# Autodesk Inventor assembly: Assembly1
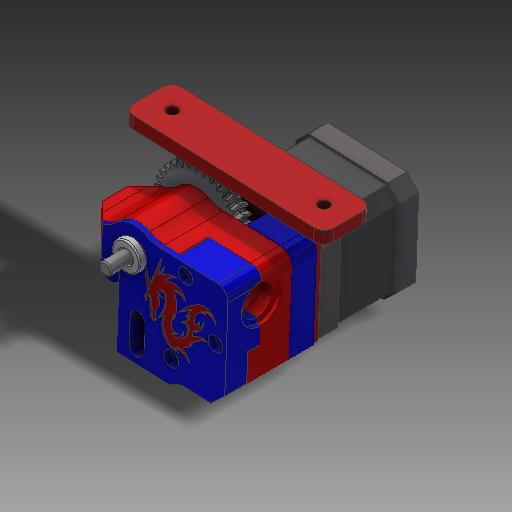
[picture p0: Inventor's stored thumbnail of the model, 512x512]
Saved by Autodesk Inventor 2017.3 (Build 213256000, 256)
## iProperties
Created: 2018-09-06
Part Number: Assembly1
Document SubType Name: Assembly
Designer: Ax
Author: Ax
## iProperties of the stored document PM Wantai 609  Nema 17.ipt
Created: 2015-03-22
Part Number: PM Wantai 609  Nema 17
Material: Generic
Document SubType Name: Modeling
Designer: Ax
Density: 1 g/cm^3
Appearance: Default
Sending System: Autodesk Inventor 2015
Preprocessor: ST-DEVELOPER v15.6
Title: D:\Dropbox\3D parts lib\Inventor\Nema 17s\Wantai 609\PM Wantai 609  Nema 17.stp
Author: Phil
## Documents named in this file (16)
- **C:\Users\Ax\Documents\Inventor\Drakon\Assembly1.iam*LocalDocs*x1hxt1kqvYop2ua0uThhu3lz2Aa*PM Wantai 609  Nema 17.ipt
- C:\Users\Ax\Documents\Inventor\Drakon\Assembly1.iam
- C:\Users\Ax\Documents\Inventor\Drakon\RAMPSDrakon_1.75_Body.ipt
- C:\Users\Ax\Documents\Inventor\Drakon\RAMPSDrakon_1.75_Cover.ipt
- C:\Users\Ax\Documents\Inventor\Drakon\RAMPSDrakon_1.75_Idler.ipt
- C:\Users\Ax\Documents\Inventor\Drakon\RAMPSDrakon_Base.ipt
- C:\Users\Ax\Documents\Inventor\Drakon\RAMPSFrame_Mount.ipt
- C:\Users\Ax\Documents\Inventor\Drakon\RAMPSDrakon_Small_Gear.ipt
- C:\Users\Ax\Documents\Inventor\Drakon\RAMPSDrakon_Large_Gear.ipt
- C:\Users\Ax\Documents\Inventor\Drakon\Library\625ZZ.ipt
- C:\Users\Ax\Documents\Inventor\Drakon\Library\M5x40_Hex_Bolt.ipt
- C:\Users\Ax\Documents\Inventor\Drakon\Library\MK8.ipt
- C:\Users\Ax\Documents\Inventor\Drakon\Library\Drakon_Spindle_Bushing.ipt
- C:\Users\Ax\Documents\Inventor\Drakon\Library\Drakon_1.75_Filament_Guide.ipt
- C:\Users\Ax\Documents\Inventor\Drakon\Assembly1\Design Accelerator\Compress Spring1.iam
- C:\Users\Ax\Documents\Git\Drakon-Extruder\FreeCAD\STEP\PM Wantai 609  Nema 17.stp
## Components (16 placed, 14 different names)
1. Drakon_1.75_Body:1 — Rigid:1, Mate:1, Mate:5, Mate:6, Rotational:4, Mate:10, Mate:11, Mate:12, Mate:13, Mate:14, Rotational:6, Mate:15, Mate:16, Mate:17, Mate:18, Mate:19, Mate:20
2. RAMPSDrakon_1.75_Cover:1 — Rigid:1, Mate:10, Mate:11, Mate:12, Cylindrical:1
3. RAMPSDrakon_1.75_Idler:1 — Rotational:4
4. RAMPSDrakon_Base:1 — Mate:1, Mate:2, Mate:4, Mate:5, Mate:6
5. PM Wantai 609  Nema 17:1 — Rotational:2, Mate:3, Mate:7, Mate:8, Mate:9, Rotational:3
6. RAMPSFrame_Mount:1 — Mate:2, Rotational:2, Mate:3, Mate:4, Mate:7, Mate:8, Mate:9
7. RAMPSDrakon_Small_Gear:1 — Rotational:3, Rotational:6
8. RAMPSDrakon_Large_Gear:1 — Rotational:7, Insert:1
9. 625ZZ:1 — Mate:14, Rotational:7, Mate:15, Rotational:8
10. 625ZZ:2 — Mate:13, Mate:16
11. M5x40_Hex_Bolt:1 — Insert:1, Rigid:2
12. MK8:1 — Rotational:8, Rotational:9
13. Drakon_Spindle_Bushing:1 — Rotational:9
14. Drakon_Spindle_Bushing:2 — Cylindrical:1, Rigid:2
15. Drakon_1.75_Filament_Guide:1 — Mate:17, Mate:18, Mate:19
16. Compress Spring:1 [sub-assembly] — Mate:20
## Relationships (31: Mate 20, RevoluteJoint 7, WeldJoint 2, Insert 1, CylindricalJoint 1)
- Rigid:1 [WeldJoint]: Drakon_1.75_Body:1 ↔ RAMPSDrakon_1.75_Cover:1
- Mate:1: Drakon_1.75_Body:1 ↔ RAMPSDrakon_Base:1
- Mate:2: RAMPSDrakon_Base:1 ↔ RAMPSFrame_Mount:1
- Rotational:2 [RevoluteJoint]: PM Wantai 609  Nema 17:1 ↔ RAMPSFrame_Mount:1
- Mate:3: PM Wantai 609  Nema 17:1 ↔ RAMPSFrame_Mount:1
- Mate:4: RAMPSDrakon_Base:1 ↔ RAMPSFrame_Mount:1
- Mate:5: Drakon_1.75_Body:1 ↔ RAMPSDrakon_Base:1
- Mate:6: Drakon_1.75_Body:1 ↔ RAMPSDrakon_Base:1
- Mate:7: PM Wantai 609  Nema 17:1 ↔ RAMPSFrame_Mount:1
- Mate:8: PM Wantai 609  Nema 17:1 ↔ RAMPSFrame_Mount:1
- Mate:9: PM Wantai 609  Nema 17:1 ↔ RAMPSFrame_Mount:1
- Rotational:3 [RevoluteJoint] (-6.35 mm): PM Wantai 609  Nema 17:1 ↔ RAMPSDrakon_Small_Gear:1
- Rotational:4 [RevoluteJoint]: Drakon_1.75_Body:1 ↔ RAMPSDrakon_1.75_Idler:1
- Mate:10: Drakon_1.75_Body:1 ↔ RAMPSDrakon_1.75_Cover:1
- Mate:11: Drakon_1.75_Body:1 ↔ RAMPSDrakon_1.75_Cover:1
- Mate:12: Drakon_1.75_Body:1 ↔ RAMPSDrakon_1.75_Cover:1
- Mate:13: Drakon_1.75_Body:1 ↔ 625ZZ:2
- Mate:14: Drakon_1.75_Body:1 ↔ 625ZZ:1
- Rotational:6 [RevoluteJoint] (-1.25 mm): Drakon_1.75_Body:1 ↔ RAMPSDrakon_Small_Gear:1
- Rotational:7 [RevoluteJoint] (-1.5 mm): RAMPSDrakon_Large_Gear:1 ↔ 625ZZ:1
- Insert:1: RAMPSDrakon_Large_Gear:1 ↔ M5x40_Hex_Bolt:1
- Mate:15: Drakon_1.75_Body:1 ↔ 625ZZ:1
- Mate:16: Drakon_1.75_Body:1 ↔ 625ZZ:2
- Rotational:8 [RevoluteJoint] (-0.75 mm): 625ZZ:1 ↔ MK8:1
- Rotational:9 [RevoluteJoint]: MK8:1 ↔ Drakon_Spindle_Bushing:1
- Cylindrical:1: RAMPSDrakon_1.75_Cover:1 ↔ Drakon_Spindle_Bushing:2
- Rigid:2 [WeldJoint] (-8.5 mm): M5x40_Hex_Bolt:1 ↔ Drakon_Spindle_Bushing:2
- Mate:17: Drakon_1.75_Body:1 ↔ Drakon_1.75_Filament_Guide:1
- Mate:18: Drakon_1.75_Body:1 ↔ Drakon_1.75_Filament_Guide:1
- Mate:19: Drakon_1.75_Body:1 ↔ Drakon_1.75_Filament_Guide:1
- Mate:20: Drakon_1.75_Body:1 ↔ Compress Spring:1
